# Autodesk Inventor assembly: Glass Door
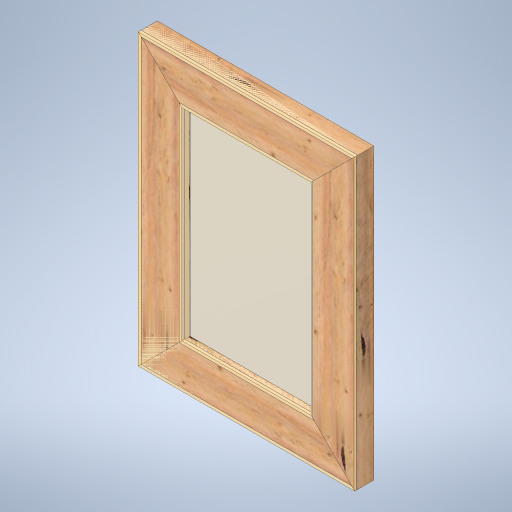
[picture p0: Inventor's stored thumbnail of the model, 512x512]
Saved by Autodesk Inventor 2024 (Build 280153000, 153)
## iProperties
RuleStatus: InUse
Created: 2014-11-18
Part Number: Glass Door
Document SubType Name: Assembly
Designer: SauliusD
Author: SauliusD
## Documents named in this file (7)
- C:\W4INV 2024 Design\iBOX LIBRARY\Facades\Glass Door\Glass Door.iam
- C:\W4INV 2024 Design\iBOX LIBRARY\Facades\Glass Door\Left Frame.ipt
- C:\W4INV 2024 Design\iBOX LIBRARY\Facades\Glass Door\Bottom Frame.ipt
- C:\W4INV 2024 Design\iBOX LIBRARY\Facades\Glass Door\Right Frame.ipt
- C:\W4INV 2024 Design\iBOX LIBRARY\Facades\Glass Door\Top frame.ipt
- C:\W4INV 2024 Design\iBOX LIBRARY\Facades\Glass Door\Glass.ipt
- C:\W4INV 2024 Design\iBOX LIBRARY\Facades\Glass Door\Glass Door.ipt
## Components (6 placed, 6 different names)
1. @Skeleton — Flush:1, Flush:2, Flush:3
2. Left Frame:1
3. Bottom Frame:1
4. Right Frame:1
5. Top frame:1
6. Glass:1
## Relationships (3: Flush 3)
- Flush:1: @Skeleton
- Flush:2: @Skeleton
- Flush:3: @Skeleton
## Named parameters: Offset_From_Left = 1.5 mm, Offset_From_Right = 1.5 mm, Offset_From_Top = 1.5 mm, Offset_From_Bottom = 1.5 mm
